# Autodesk Inventor assembly: Clamp with Piston Assembly
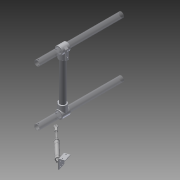
[picture p0: Inventor's stored thumbnail of the model, 180x180]
Saved by Autodesk Inventor 2014 (Build 180170000, 170)
## iProperties
Created: 2014-01-12
Part Number: Clamp with Piston Assembly
Document SubType Name: Assembly
Designer: Michael
Mass: 305.276 g
Surface Area: 1793.78 cm^2
Volume: 181.752 cm^3
Density: 1.67964 g/cm^3
Author: Michael
## Documents named in this file (5)
- C:\Users\Michael\Documents\GitHub\2014buildCAD\Collector\Clamp with Piston Assembly.iam
- C:\Users\Michael\Documents\GitHub\2014buildCAD\Collector\Polycarbonate Clamp Tube (Middle) (8585K14).ipt
- C:\Users\Michael\Documents\GitHub\2014buildCAD\Collector\Polycarbonate Clamp Tube 1 in OD (8585K14).ipt
- C:\Users\Michael\Documents\GitHub\2014buildCAD\Collector\Metal Pipe T Joint (4698T140).ipt
- C:\Users\Michael\Documents\GitHub\2014buildCAD\Collector\Piston Assembly.iam
## Components (6 placed, 4 different names)
1. Polycarbonate Clamp Tube (Middle) (8585K14):1 — Mate:3, Mate:4, Mate:5, Mate:6
2. Polycarbonate Clamp Tube 1 in OD (8585K14):1 — Mate:1, Flush:1, Angle:1, Mate:7
3. Polycarbonate Clamp Tube 1 in OD (8585K14):2 — Mate:2, Flush:2, Angle:1, Mate:8
4. Metal Pipe T Joint (4698T140):1 — Mate:1, Flush:1, Mate:3, Mate:5
5. Metal Pipe T Joint (4698T140):2 — Mate:2, Flush:2, Mate:4, Mate:6
6. Piston Assembly:2 [sub-assembly] — Mate:7, Mate:8
## Relationships (11: Mate 8, Flush 2, Angle 1)
- Mate:1: Polycarbonate Clamp Tube 1 in OD (8585K14):1 ↔ Metal Pipe T Joint (4698T140):1
- Flush:1 (101.6 mm): Polycarbonate Clamp Tube 1 in OD (8585K14):1 ↔ Metal Pipe T Joint (4698T140):1
- Mate:2: Polycarbonate Clamp Tube 1 in OD (8585K14):2 ↔ Metal Pipe T Joint (4698T140):2
- Flush:2 (101.6 mm): Polycarbonate Clamp Tube 1 in OD (8585K14):2 ↔ Metal Pipe T Joint (4698T140):2
- Mate:3: Polycarbonate Clamp Tube (Middle) (8585K14):1 ↔ Metal Pipe T Joint (4698T140):1
- Mate:4: Polycarbonate Clamp Tube (Middle) (8585K14):1 ↔ Metal Pipe T Joint (4698T140):2
- Mate:5 (-23.8125 mm): Polycarbonate Clamp Tube (Middle) (8585K14):1 ↔ Metal Pipe T Joint (4698T140):1
- Mate:6 (-23.8125 mm): Polycarbonate Clamp Tube (Middle) (8585K14):1 ↔ Metal Pipe T Joint (4698T140):2
- Angle:1 (0 deg): Polycarbonate Clamp Tube 1 in OD (8585K14):1 ↔ Polycarbonate Clamp Tube 1 in OD (8585K14):2
- Mate:7: Polycarbonate Clamp Tube 1 in OD (8585K14):1 ↔ Piston Assembly:2
- Mate:8 (38.1 mm): Polycarbonate Clamp Tube 1 in OD (8585K14):2 ↔ Piston Assembly:2
